# Autodesk Inventor assembly: Assembly1
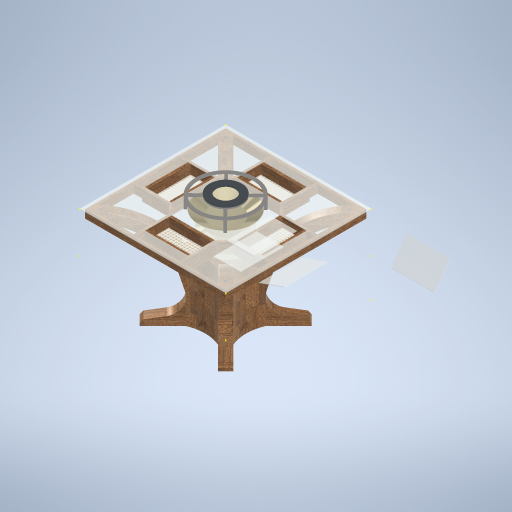
[picture p0: Inventor's stored thumbnail of the model, 512x512]
Saved by Autodesk Inventor 2023 (Build 270158000, 158)
## iProperties
Created: 2022-11-22
Part Number: Assembly1
Document SubType Name: Assembly
Designer: surat
Author: surat
## Documents named in this file (17)
- C:\Users\surat\Documents\Table project\Assembly1.iam
- C:\Users\surat\Documents\Table project\Main frame Piece X4.ipt
- C:\Users\surat\Documents\Table project\Secondary frame for drawrs long piece X8.ipt
- C:\Users\surat\Documents\Table project\Tall drawn wall.ipt
- C:\Users\surat\Documents\Table project\angle interior piece X4.ipt
- C:\Users\surat\Documents\Table project\Glass top X1.ipt
- C:\Users\surat\Documents\Table project\glass holder drawr X8.ipt
- C:\Users\surat\Documents\Table project\glass bottem container X4.ipt
- C:\Users\surat\Documents\Table project\Table Leg X4.ipt
- C:\Users\surat\Documents\Table project\Table Base X1.ipt
- C:\Users\surat\Documents\Table project\Table foot X4.ipt
- C:\Users\surat\Documents\Table project\Mesh under bins X4.ipt
- C:\Users\surat\Documents\Table project\Glass panal for the opening X4.ipt
- C:\Users\surat\Documents\Table project\Trash bin casing X1.ipt
- C:\Users\surat\Documents\Table project\Glass mount X4.ipt
- C:\Users\surat\Documents\Table project\Lazy suzan lower frame.ipt
- C:\Users\surat\Documents\Table project\Mock Bearing X1.ipt
## Components (61 placed, 16 different names)
1. Main frame Piece X4:1 — Mate:1, Flush:1, Mate:2, Flush:3, Insert:7, Flush:10, Insert:8, Flush:11, Mate:45, Mate:50, Flush:29
2. Main frame Piece X4:2 — Mate:1, Flush:1, Mate:2, Mate:3, Flush:2, Mate:4, Insert:1, Flush:4, Insert:2, Flush:5, Mate:51, Mate:54, Flush:32
3. Main frame Piece X4:3 — Mate:3, Flush:2, Mate:4, Mate:5, Mate:6, Insert:3, Flush:6, Insert:4, Flush:7, Mate:48, Mate:53, Flush:30, Flush:33
4. Main frame Piece X4:4 — Mate:5, Flush:3, Mate:6, Insert:5, Flush:8, Flush:9, Insert:6, Mate:44, Mate:47, Flush:28, Flush:31
5. Secondary frame for drawrs long piece X8:1 — Insert:8, Flush:11, Insert:21, Mate:30
6. Secondary frame for drawrs long piece X8:2 — Insert:7, Flush:10, Insert:11, Flush:14, Insert:16, Flush:19, Mate:9
7. Secondary frame for drawrs long piece X8:3 — Insert:2, Flush:5, Insert:17, Flush:23, Mate:21
8. Secondary frame for drawrs long piece X8:4 — Insert:3, Flush:6, Insert:10, Flush:13, Flush:20, Insert:19, Mate:24
9. Secondary frame for drawrs long piece X8:5 — Insert:5, Flush:8, Insert:12, Flush:15, Insert:14, Flush:17, Insert:20, Mate:18
10. Secondary frame for drawrs long piece X8:6 — Flush:9, Insert:6, Insert:15, Flush:18, Mate:27
11. Secondary frame for drawrs long piece X8:7 — Insert:1, Flush:4, Insert:13, Flush:16, Insert:18, Mate:12
12. Secondary frame for drawrs long piece X8:8 — Insert:4, Flush:7, Flush:24, Mate:15
13. Tall drawn wall:1 — Insert:11, Flush:14, Flush:26, Mate:31, Mate:43
14. Tall drawn wall:2 — Insert:10, Flush:13, Mate:25, Mate:72
15. Tall drawn wall:3 — Insert:12, Flush:15, Flush:25, Mate:19, Mate:28, Mate:34, Mate:62
16. Tall drawn wall:4 — Insert:13, Flush:16, Mate:11, Mate:22, Mate:40, Mate:68
17. angle interior piece X4:1 — Insert:14, Flush:17
18. angle interior piece X4:2 — Insert:15, Flush:18
19. angle interior piece X4:3 — Insert:16, Flush:19
20. angle interior piece X4:4 — Insert:17, Flush:20
21. Tall drawn wall:5 — Insert:18, Flush:23, Mate:13, Mate:20
22. Tall drawn wall:6 — Insert:21, Flush:26, Mate:8, Mate:10, Mate:29, Mate:65
23. Tall drawn wall:7 — Insert:20, Flush:25, Mate:17, Mate:26
24. Tall drawn wall:8 — Insert:19, Flush:24, Mate:14, Mate:16, Mate:23, Mate:37
25. glass holder drawr X8:1 — Mate:14, Mate:15, Mate:16, Mate:35
26. glass holder drawr X8:2 — Mate:26, Mate:27, Mate:28
27. glass holder drawr X8:3 — Mate:20, Mate:21, Mate:22, Mate:38, Mate:69
28. glass holder drawr X8:4 — Mate:23, Mate:24, Mate:25, Mate:36, Mate:71
29. glass holder drawr X8:5 — Mate:29, Mate:30, Mate:31, Mate:41
30. glass holder drawr X8:6 — Mate:17, Mate:18, Mate:19, Mate:32, Mate:33, Mate:63
31. glass holder drawr X8:7 — Mate:11, Mate:12, Mate:13, Mate:39
32. glass holder drawr X8:8 — Mate:8, Mate:9, Mate:10, Mate:42, Mate:66
33. glass bottem container X4:1 — Mate:32, Mate:33, Mate:34, Mate:61
34. glass bottem container X4:2 — Mate:35, Mate:36, Mate:37, Mate:70
35. glass bottem container X4:3 — Mate:38, Mate:39, Mate:40, Mate:67
36. glass bottem container X4:4 — Mate:41, Mate:42, Mate:43, Mate:64
37. Table Leg X4:1 — Mate:47, Mate:48, Mate:56, Flush:31, Mate:82, Mate:83
38. Table Leg X4:2 — Mate:53, Mate:54, Insert:22, Flush:30, Mate:84, Mate:85
39. Table Leg X4:3 — Mate:50, Mate:51, Flush:29, Mate:80, Mate:81
40. Table Leg X4:4 — Mate:44, Mate:45, Mate:78, Mate:79, Flush:28
41. Table Base X1:1 — Insert:22, Mate:56, Insert:23, Mate:57, Insert:24, Mate:58, Insert:25, Mate:59, Insert:26, Mate:60, Mate:77, Flush:27
42. Table foot X4:1 — Insert:26, Mate:60
43. Table foot X4:2 — Insert:25, Mate:59
44. Table foot X4:3 — Insert:24, Mate:58
45. Table foot X4:4 — Insert:23, Mate:57
46. Mesh under bins X4:1 — Mate:70, Mate:71, Mate:72
47. Mesh under bins X4:2 — Mate:67, Mate:68, Mate:69
48. Mesh under bins X4:3 — Mate:64, Mate:65, Mate:66
49. Mesh under bins X4:4 — Mate:61, Mate:62, Mate:63
50. Glass panal for the opening X4:2
51. Glass panal for the opening X4:3
52. Glass panal for the opening X4:4
53. Glass panal for the opening X4:5
54. Trash bin casing X1:1 — Mate:77, Flush:27, Mate:87
55. Glass mount X4:1 — Mate:80, Mate:81
56. Glass mount X4:2 — Mate:84, Mate:85, Mate:86
57. Glass mount X4:3 — Mate:82, Mate:83
58. Glass mount X4:4 — Mate:78, Mate:79
59. Glass top X1:1 — Mate:86, Flush:32, Flush:33, Mate:88
60. Lazy suzan lower frame:1 — Mate:87, Mate:88, Mate:89, Insert:27
61. Mock Bearing X1:1 — Mate:89, Insert:27
## Relationships (136: Mate 80, Flush 30, Insert 26)
- Mate:1: Main frame Piece X4:1 ↔ Main frame Piece X4:2
- Flush:1: Main frame Piece X4:1 ↔ Main frame Piece X4:2
- Mate:2: Main frame Piece X4:1 ↔ Main frame Piece X4:2
- Mate:3: Main frame Piece X4:2 ↔ Main frame Piece X4:3
- Flush:2: Main frame Piece X4:2 ↔ Main frame Piece X4:3
- Mate:4: Main frame Piece X4:2 ↔ Main frame Piece X4:3
- Mate:5: Main frame Piece X4:3 ↔ Main frame Piece X4:4
- Flush:3: Main frame Piece X4:1 ↔ Main frame Piece X4:4
- Mate:6: Main frame Piece X4:3 ↔ Main frame Piece X4:4
- Insert:1: Main frame Piece X4:2 ↔ Secondary frame for drawrs long piece X8:7
- Flush:4: Main frame Piece X4:2 ↔ Secondary frame for drawrs long piece X8:7
- Insert:2: Main frame Piece X4:2 ↔ Secondary frame for drawrs long piece X8:3
- Flush:5: Main frame Piece X4:2 ↔ Secondary frame for drawrs long piece X8:3
- Insert:3: Main frame Piece X4:3 ↔ Secondary frame for drawrs long piece X8:4
- Flush:6: Main frame Piece X4:3 ↔ Secondary frame for drawrs long piece X8:4
- Insert:4: Main frame Piece X4:3 ↔ Secondary frame for drawrs long piece X8:8
- Flush:7: Main frame Piece X4:3 ↔ Secondary frame for drawrs long piece X8:8
- Insert:5: Main frame Piece X4:4 ↔ Secondary frame for drawrs long piece X8:5
- Flush:8: Main frame Piece X4:4 ↔ Secondary frame for drawrs long piece X8:5
- Flush:9: Main frame Piece X4:4 ↔ Secondary frame for drawrs long piece X8:6
- Insert:6: Main frame Piece X4:4 ↔ Secondary frame for drawrs long piece X8:6
- Insert:7: Main frame Piece X4:1 ↔ Secondary frame for drawrs long piece X8:2
- Flush:10: Main frame Piece X4:1 ↔ Secondary frame for drawrs long piece X8:2
- Insert:8: Main frame Piece X4:1 ↔ Secondary frame for drawrs long piece X8:1
- Flush:11: Main frame Piece X4:1 ↔ Secondary frame for drawrs long piece X8:1
- Insert:10: Secondary frame for drawrs long piece X8:4 ↔ Tall drawn wall:2
- Flush:13: Secondary frame for drawrs long piece X8:4 ↔ Tall drawn wall:2
- Insert:11: Secondary frame for drawrs long piece X8:2 ↔ Tall drawn wall:1
- Flush:14: Secondary frame for drawrs long piece X8:2 ↔ Tall drawn wall:1
- Insert:12: Secondary frame for drawrs long piece X8:5 ↔ Tall drawn wall:3
- Flush:15: Secondary frame for drawrs long piece X8:5 ↔ Tall drawn wall:3
- Insert:13: Secondary frame for drawrs long piece X8:7 ↔ Tall drawn wall:4
- Flush:16: Secondary frame for drawrs long piece X8:7 ↔ Tall drawn wall:4
- Insert:14: Secondary frame for drawrs long piece X8:5 ↔ angle interior piece X4:1
- Flush:17: Secondary frame for drawrs long piece X8:5 ↔ angle interior piece X4:1
- Insert:15: Secondary frame for drawrs long piece X8:6 ↔ angle interior piece X4:2
- Flush:18: Secondary frame for drawrs long piece X8:6 ↔ angle interior piece X4:2
- Insert:16: Secondary frame for drawrs long piece X8:2 ↔ angle interior piece X4:3
- Flush:19: Secondary frame for drawrs long piece X8:2 ↔ angle interior piece X4:3
- Insert:17: Secondary frame for drawrs long piece X8:3 ↔ angle interior piece X4:4
- Flush:20: Secondary frame for drawrs long piece X8:4 ↔ angle interior piece X4:4
- Insert:18: Secondary frame for drawrs long piece X8:7 ↔ Tall drawn wall:5
- Flush:23 (25.4 mm): Secondary frame for drawrs long piece X8:3 ↔ Tall drawn wall:5
- Insert:19: Secondary frame for drawrs long piece X8:4 ↔ Tall drawn wall:8
- Flush:24 (25.4 mm): Secondary frame for drawrs long piece X8:8 ↔ Tall drawn wall:8
- Insert:20: Secondary frame for drawrs long piece X8:5 ↔ Tall drawn wall:7
- Flush:25: Tall drawn wall:3 ↔ Tall drawn wall:7
- Insert:21: Secondary frame for drawrs long piece X8:1 ↔ Tall drawn wall:6
- Flush:26: Tall drawn wall:1 ↔ Tall drawn wall:6
- Mate:8: Tall drawn wall:6 ↔ glass holder drawr X8:8
- Mate:9: Secondary frame for drawrs long piece X8:2 ↔ glass holder drawr X8:8
- Mate:10: Tall drawn wall:6 ↔ glass holder drawr X8:8
- Mate:11: Tall drawn wall:4 ↔ glass holder drawr X8:7
- Mate:12: Secondary frame for drawrs long piece X8:7 ↔ glass holder drawr X8:7
- Mate:13: Tall drawn wall:5 ↔ glass holder drawr X8:7
- Mate:14: Tall drawn wall:8 ↔ glass holder drawr X8:1
- Mate:15: Secondary frame for drawrs long piece X8:8 ↔ glass holder drawr X8:1
- Mate:16: Tall drawn wall:8 ↔ glass holder drawr X8:1
- Mate:17: Tall drawn wall:7 ↔ glass holder drawr X8:6
- Mate:18: Secondary frame for drawrs long piece X8:5 ↔ glass holder drawr X8:6
- Mate:19: Tall drawn wall:3 ↔ glass holder drawr X8:6
- Mate:20: Tall drawn wall:5 ↔ glass holder drawr X8:3
- Mate:21: Secondary frame for drawrs long piece X8:3 ↔ glass holder drawr X8:3
- Mate:22: Tall drawn wall:4 ↔ glass holder drawr X8:3
- Mate:23: Tall drawn wall:8 ↔ glass holder drawr X8:4
- Mate:24: Secondary frame for drawrs long piece X8:4 ↔ glass holder drawr X8:4
- Mate:25: Tall drawn wall:2 ↔ glass holder drawr X8:4
- Mate:26: Tall drawn wall:7 ↔ glass holder drawr X8:2
- Mate:27: Secondary frame for drawrs long piece X8:6 ↔ glass holder drawr X8:2
- Mate:28: Tall drawn wall:3 ↔ glass holder drawr X8:2
- Mate:29: Tall drawn wall:6 ↔ glass holder drawr X8:5
- Mate:30: Secondary frame for drawrs long piece X8:1 ↔ glass holder drawr X8:5
- Mate:31: Tall drawn wall:1 ↔ glass holder drawr X8:5
- Mate:32: glass holder drawr X8:6 ↔ glass bottem container X4:1
- Mate:33: glass holder drawr X8:6 ↔ glass bottem container X4:1
- Mate:34: Tall drawn wall:3 ↔ glass bottem container X4:1
- Mate:35: glass holder drawr X8:1 ↔ glass bottem container X4:2
- Mate:36: glass holder drawr X8:4 ↔ glass bottem container X4:2
- Mate:37: Tall drawn wall:8 ↔ glass bottem container X4:2
- Mate:38: glass holder drawr X8:3 ↔ glass bottem container X4:3
- Mate:39: glass holder drawr X8:7 ↔ glass bottem container X4:3
- Mate:40: Tall drawn wall:4 ↔ glass bottem container X4:3
- Mate:41: glass holder drawr X8:5 ↔ glass bottem container X4:4
- Mate:42: glass holder drawr X8:8 ↔ glass bottem container X4:4
- Mate:43: Tall drawn wall:1 ↔ glass bottem container X4:4
- Mate:44: Main frame Piece X4:4 ↔ Table Leg X4:4
- Mate:45: Main frame Piece X4:1 ↔ Table Leg X4:4
- Mate:47: Main frame Piece X4:4 ↔ Table Leg X4:1
- Mate:48: Main frame Piece X4:3 ↔ Table Leg X4:1
- Mate:50: Main frame Piece X4:1 ↔ Table Leg X4:3
- Mate:51: Main frame Piece X4:2 ↔ Table Leg X4:3
- Mate:53: Main frame Piece X4:3 ↔ Table Leg X4:2
- Mate:54: Main frame Piece X4:2 ↔ Table Leg X4:2
- Insert:22: Table Leg X4:2 ↔ Table Base X1:1
- Mate:56: Table Leg X4:1 ↔ Table Base X1:1
- Insert:23: Table Base X1:1 ↔ Table foot X4:4
- Mate:57: Table Base X1:1 ↔ Table foot X4:4
- Insert:24: Table Base X1:1 ↔ Table foot X4:3
- Mate:58: Table Base X1:1 ↔ Table foot X4:3
- Insert:25: Table Base X1:1 ↔ Table foot X4:2
- Mate:59: Table Base X1:1 ↔ Table foot X4:2
- Insert:26: Table Base X1:1 ↔ Table foot X4:1
- Mate:60: Table Base X1:1 ↔ Table foot X4:1
- Mate:61: glass bottem container X4:1 ↔ Mesh under bins X4:4
- Mate:62: Tall drawn wall:3 ↔ Mesh under bins X4:4
- Mate:63: glass holder drawr X8:6 ↔ Mesh under bins X4:4
- Mate:64: glass bottem container X4:4 ↔ Mesh under bins X4:3
- Mate:65: Tall drawn wall:6 ↔ Mesh under bins X4:3
- Mate:66: glass holder drawr X8:8 ↔ Mesh under bins X4:3
- Mate:67: glass bottem container X4:3 ↔ Mesh under bins X4:2
- Mate:68: Tall drawn wall:4 ↔ Mesh under bins X4:2
- Mate:69: glass holder drawr X8:3 ↔ Mesh under bins X4:2
- Mate:70: glass bottem container X4:2 ↔ Mesh under bins X4:1
- Mate:71: glass holder drawr X8:4 ↔ Mesh under bins X4:1
- Mate:72: Tall drawn wall:2 ↔ Mesh under bins X4:1
- Mate:77: Table Base X1:1 ↔ Trash bin casing X1:1
- Flush:27: Table Base X1:1 ↔ Trash bin casing X1:1
- Mate:78: Table Leg X4:4 ↔ Glass mount X4:4
- Mate:79: Table Leg X4:4 ↔ Glass mount X4:4
- Flush:28: Main frame Piece X4:4 ↔ Table Leg X4:4
- Flush:29: Main frame Piece X4:1 ↔ Table Leg X4:3
- Flush:30: Main frame Piece X4:3 ↔ Table Leg X4:2
- Flush:31: Main frame Piece X4:4 ↔ Table Leg X4:1
- Mate:80: Table Leg X4:3 ↔ Glass mount X4:1
- Mate:81: Table Leg X4:3 ↔ Glass mount X4:1
- Mate:82: Table Leg X4:1 ↔ Glass mount X4:3
- Mate:83: Table Leg X4:1 ↔ Glass mount X4:3
- Mate:84: Table Leg X4:2 ↔ Glass mount X4:2
- Mate:85: Table Leg X4:2 ↔ Glass mount X4:2
- Mate:86: Glass mount X4:2 ↔ Glass top X1:1
- Flush:32 (25.4 mm): Main frame Piece X4:2 ↔ Glass top X1:1
- Flush:33 (25.4 mm): Main frame Piece X4:3 ↔ Glass top X1:1
- Mate:87: Trash bin casing X1:1 ↔ Lazy suzan lower frame:1
- Mate:88: Glass top X1:1 ↔ Lazy suzan lower frame:1
- Mate:89: Lazy suzan lower frame:1 ↔ Mock Bearing X1:1
- Insert:27: Lazy suzan lower frame:1 ↔ Mock Bearing X1:1
